# Autodesk Inventor assembly: vert_motor_mount
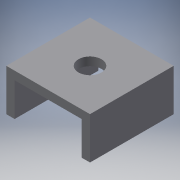
[picture p0: Inventor's stored thumbnail of the model, 180x180]
Saved by Autodesk Inventor 2019 (Build 230136000, 136)
## iProperties
Created: 2018-12-13
Part Number: vert_motor_mount
Document SubType Name: Assembly
Designer: garstka1245
Author: garstka1245
## Documents named in this file (3)
- H:\Engineering Club\Vert motor mount\vert_motor_mount.iam
- H:\Engineering Club\Vert motor mount\base.ipt
- H:\Engineering Club\Vert motor mount\side.ipt
## Components (3 placed, 2 different names)
1. base:1 — Mate:1, Mate:2, Flush:1, Flush:2, Flush:3, Flush:4
2. side:1 — Mate:2, Flush:1, Flush:4
3. side:2 — Mate:1, Flush:2, Flush:3
## Relationships (6: Flush 4, Mate 2)
- Mate:1: base:1 ↔ side:2
- Mate:2: base:1 ↔ side:1
- Flush:1: base:1 ↔ side:1
- Flush:2: base:1 ↔ side:2
- Flush:3: base:1 ↔ side:2
- Flush:4: base:1 ↔ side:1
